# Autodesk Inventor assembly: 대충조립품1
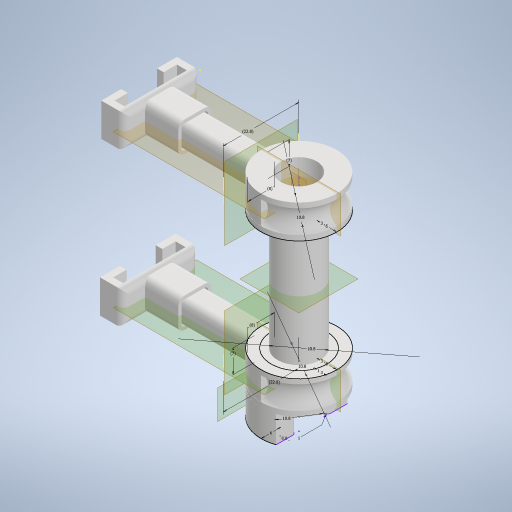
[picture p0: Inventor's stored thumbnail of the model, 512x512]
Saved by Autodesk Inventor 2023 (Build 270158000, 158)
## iProperties
Created: 2023-04-26
Part Number: 대충조립품1
Document SubType Name: Assembly
Designer: rlatk
Author: rlatk
## Documents named in this file (6)
- C:\Users\rlatk\Desktop\코일건\코일건 부품\대충조립품1.iam
- C:\Users\rlatk\Desktop\코일건\코일건 부품\코일감는부분1.ipt
- C:\Users\rlatk\Desktop\코일건\코일건 부품\코일건원통꼽게1.ipt
- C:\Users\rlatk\Desktop\코일건\코일건 부품\ir다이오드4.ipt
- C:\Users\rlatk\Desktop\코일건\코일건 부품\막대2.ipt
- C:\Users\rlatk\Desktop\코일건\코일건 부품\막대꼽게1.ipt
## Components (8 placed, 5 different names)
1. 코일감는부분1:1 — 회전:1, 회전:2
2. 코일건원통꼽게1:1 — 회전:1, 강체:2
3. 코일건원통꼽게1:2 — 회전:2, 회전:3, 강체:1
4. ir다이오드4:1 — 회전:3
5. 막대2:1 — 강체:1, 강체:3
6. 막대2:2 — 강체:2, 강체:4
7. 막대꼽게1:1 — 강체:3
8. 막대꼽게1:2 — 강체:4
## Relationships (7: WeldJoint 4, RevoluteJoint 3)
- 회전:1 [RevoluteJoint]: 코일감는부분1:1 ↔ 코일건원통꼽게1:1
- 회전:2 [RevoluteJoint]: 코일감는부분1:1 ↔ 코일건원통꼽게1:2
- 회전:3 [RevoluteJoint]: 코일건원통꼽게1:2 ↔ ir다이오드4:1
- 강체:1 [WeldJoint]: 코일건원통꼽게1:2 ↔ 막대2:1
- 강체:2 [WeldJoint]: 코일건원통꼽게1:1 ↔ 막대2:2
- 강체:3 [WeldJoint]: 막대2:1 ↔ 막대꼽게1:1
- 강체:4 [WeldJoint]: 막대2:2 ↔ 막대꼽게1:2
